# Autodesk Inventor assembly: Tafe Wa Logo
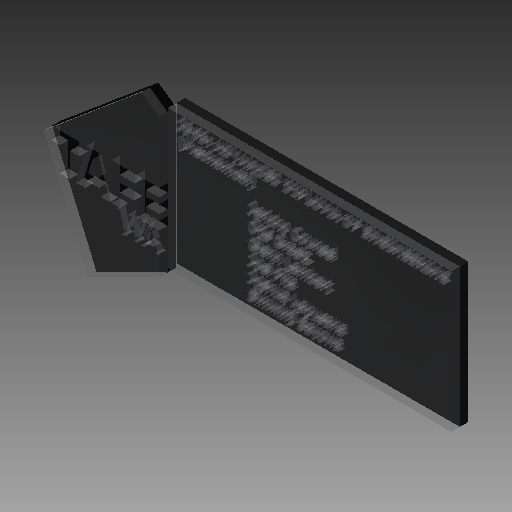
[picture p0: Inventor's stored thumbnail of the model, 512x512]
Saved by Autodesk Inventor 2018 (Build 220112000, 112)
## iProperties
Created: 2018-10-30
Part Number: Tafe Wa Logo
Document SubType Name: Assembly
Designer: Otis PC
Author: Otis PC
## Documents named in this file (5)
- C:\Users\M201291\Documents\GitHub\CNC-Lathe-CAD\CNC Lathe Project\Project Files\LOGO\Tafe Wa Logo.iam
- C:\Users\M201291\Documents\GitHub\CNC-Lathe-CAD\CNC Lathe Project\Project Files\LOGO\Tage logo 2,0.ipt
- C:\Users\M201291\Documents\GitHub\CNC-Lathe-CAD\CNC Lathe Project\Project Files\LOGO\Tafe WA LOGO backplate.ipt
- C:\Users\M201291\Documents\GitHub\CNC-Lathe-CAD\CNC Lathe Project\Project Files\LOGO\Group Name Plate back plate.ipt
- C:\Users\M201291\Documents\GitHub\CNC-Lathe-CAD\CNC Lathe Project\Project Files\LOGO\Group Name Plate.ipt
## Components (4 placed, 4 different names)
1. Tage logo 2,0:1 — Mate:1, Mate:2, Mate:3
2. Tafe WA LOGO backplate:1 — Mate:1, Mate:2, Mate:3
3. Group Name Plate back plate:1 — Mate:4, Mate:5, Mate:6
4. Group Name Plate:1 — Mate:4, Mate:5, Mate:6
## Relationships (6: Mate 6)
- Mate:1: Tage logo 2,0:1 ↔ Tafe WA LOGO backplate:1
- Mate:2: Tage logo 2,0:1 ↔ Tafe WA LOGO backplate:1
- Mate:3: Tage logo 2,0:1 ↔ Tafe WA LOGO backplate:1
- Mate:4: Group Name Plate back plate:1 ↔ Group Name Plate:1
- Mate:5: Group Name Plate back plate:1 ↔ Group Name Plate:1
- Mate:6: Group Name Plate back plate:1 ↔ Group Name Plate:1
